# Autodesk Inventor assembly: Test3
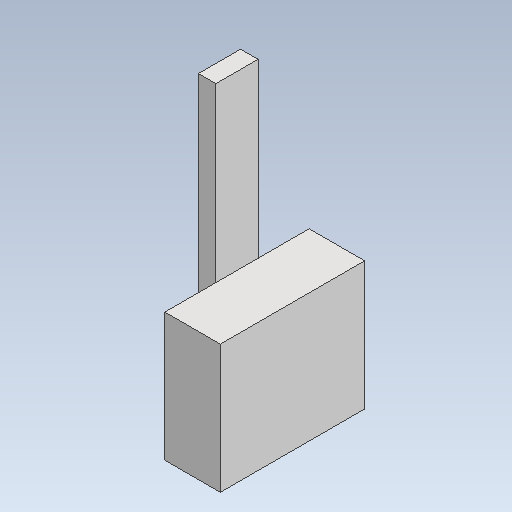
[picture p0: Inventor's stored thumbnail of the model, 512x512]
Saved by Autodesk Inventor 2025.2 (Build 292293000, 293)
## iProperties
Created: 2025-05-19
Part Number: Test3
Document SubType Name: Assembly
Designer: Sergio Quintero
Mass: 64100 g
Surface Area: 12156.5 cm^2
Volume: 55282 cm^3
Density: 1.15951 g/cm^3
Author: Sergio Quintero
## Documents named in this file (3)
- C:\Users\Sergio Quintero\OneDrive - Universidad Nacional de Colombia\Keio University\Thesis\CAD\Ball_screw\Test3.iam
- C:\Users\Sergio Quintero\OneDrive - Universidad Nacional de Colombia\Keio University\Thesis\CAD\Ball_screw\Test1.ipt
- C:\Users\Sergio Quintero\OneDrive - Universidad Nacional de Colombia\Keio University\Thesis\CAD\Ball_screw\Test2.ipt
## Components (2 placed, 2 different names)
1. Test1:1 — Rigid:1
2. Test2:1 — Rigid:1
## Relationships (1: WeldJoint 1)
- Rigid:1 [WeldJoint] (-129 mm): Test1:1 ↔ Test2:1
